# Autodesk Inventor assembly: SpurGearsFeeder
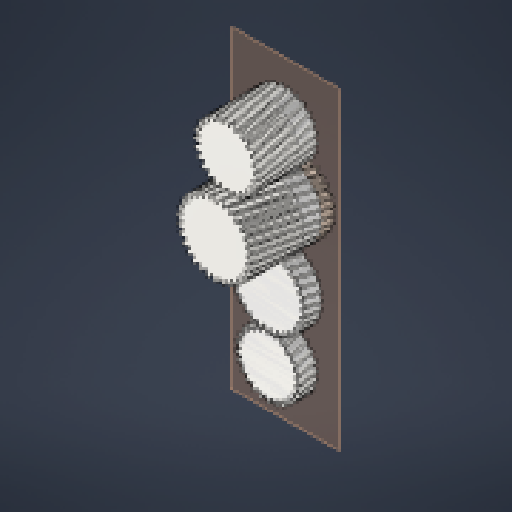
[picture p0: Inventor's stored thumbnail of the model, 512x512]
Saved by Autodesk Inventor 2024.3 (Build 283343000, 343)
## iProperties
Created: 2025-03-10
Part Number: SpurGearsFeeder
Document SubType Name: Assembly
Designer: jings
Author: jings
## Documents named in this file (4)
- C:\Users\jings\OneDrive\Desktop\2025-Poseidon-Mechanical\SpurGearsFeeder.iam
- C:\Users\jings\OneDrive\Desktop\2025-Poseidon-Mechanical\gearTemplate.ipt
- C:\Users\jings\OneDrive\Desktop\2025-Poseidon-Mechanical\SpurGearsFeeder\Design Accelerator\Spur Gears1.iam
- C:\Users\jings\OneDrive\Desktop\2025-Poseidon-Mechanical\SpurGearsFeeder\Design Accelerator\Spur Gears2.iam
## Components (3 placed, 2 different names)
1. gearTemplate:1 — Mate:5, Flush:3, Mate:6, Flush:4, Mate:7, Flush:5, Mate:8, Flush:6
2. Spur Gears:1 [sub-assembly] — Mate:5, Flush:3, Mate:6, Flush:4
3. Spur Gears:2 [sub-assembly] — Mate:7, Flush:5, Mate:8, Flush:6
## Relationships (8: Mate 4, Flush 4)
- Mate:5: gearTemplate:1 ↔ Spur Gears:1
- Flush:3: gearTemplate:1 ↔ Spur Gears:1
- Mate:6: gearTemplate:1 ↔ Spur Gears:1
- Flush:4: gearTemplate:1 ↔ Spur Gears:1
- Mate:7: gearTemplate:1 ↔ Spur Gears:2
- Flush:5: gearTemplate:1 ↔ Spur Gears:2
- Mate:8: gearTemplate:1 ↔ Spur Gears:2
- Flush:6: gearTemplate:1 ↔ Spur Gears:2
